# Autodesk Inventor assembly: Health_module_contactBoard
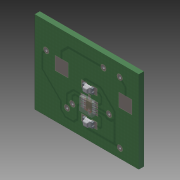
[picture p0: Inventor's stored thumbnail of the model, 180x180]
Saved by Autodesk Inventor 2013 (Build 170138000, 138)
## iProperties
Created: 2015-07-04
Part Number: Health_module_contactBoard
Document SubType Name: Assembly
Designer: terg
Author: terg
## Documents named in this file (6)
- C:\Users\terg\Projects\ModularElectronics\3D_models\Health_module\Health_module_contactBoard.iam
- C:\Users\terg\Projects\ModularElectronics\3D_models\Health_module\Health_module_contactBoard.ipt
- C:\Users\terg\Projects\ModularElectronics\3D_models\Components\0603_led.ipt
- C:\Users\terg\Projects\ModularElectronics\3D_models\Sensor_module\Si1143.ipt
- C:\Users\terg\Projects\ModularElectronics\3D_models\Components\0402_cap.ipt
- C:\Users\terg\Projects\ModularElectronics\3D_models\Components\0805_cap.ipt
## Components (6 placed, 5 different names)
1. Health_module_contactBoard:1 — Zestawiający:1, Zestawiający:2, Zestawiający:3, Równoległy:1, Równoległy:2, Równoległy:3, Równoległy:4, Równoległy:5, Równoległy:6, Zestawiający:4, Zestawiający:5, Równoległy:7, Równoległy:8, Równoległy:9, Równoległy:10
2. 0603_led:1 — Zestawiający:1, Równoległy:1, Równoległy:4
3. 0603_led:2 — Zestawiający:2, Równoległy:3, Równoległy:6
4. Si1143:1 — Zestawiający:3, Równoległy:2, Równoległy:5
5. 0402_cap:1 — Zestawiający:5, Równoległy:8, Równoległy:9
6. 0805_cap:1 — Zestawiający:4, Równoległy:7, Równoległy:10
## Relationships (15: Flush 10, Mate 5)
- Zestawiający:1 [Mate]: Health_module_contactBoard:1 ↔ 0603_led:1
- Zestawiający:2 [Mate]: Health_module_contactBoard:1 ↔ 0603_led:2
- Zestawiający:3 [Mate]: Health_module_contactBoard:1 ↔ Si1143:1
- Równoległy:1 [Flush] (2.222 mm): Health_module_contactBoard:1 ↔ 0603_led:1
- Równoległy:2 [Flush] (3.972 mm): Health_module_contactBoard:1 ↔ Si1143:1
- Równoległy:3 [Flush] (6.849 mm): Health_module_contactBoard:1 ↔ 0603_led:2
- Równoległy:4 [Flush] (7.825 mm): Health_module_contactBoard:1 ↔ 0603_led:1
- Równoległy:5 [Flush] (7.64 mm): Health_module_contactBoard:1 ↔ Si1143:1
- Równoległy:6 [Flush] (7.809 mm): Health_module_contactBoard:1 ↔ 0603_led:2
- Zestawiający:4 [Mate]: Health_module_contactBoard:1 ↔ 0805_cap:1
- Zestawiający:5 [Mate]: Health_module_contactBoard:1 ↔ 0402_cap:1
- Równoległy:7 [Flush] (3.182 mm): Health_module_contactBoard:1 ↔ 0805_cap:1
- Równoległy:8 [Flush] (3.729 mm): Health_module_contactBoard:1 ↔ 0402_cap:1
- Równoległy:9 [Flush] (3.012 mm): Health_module_contactBoard:1 ↔ 0402_cap:1
- Równoległy:10 [Flush] (4.104 mm): Health_module_contactBoard:1 ↔ 0805_cap:1
